# Autodesk Inventor assembly: entire arm
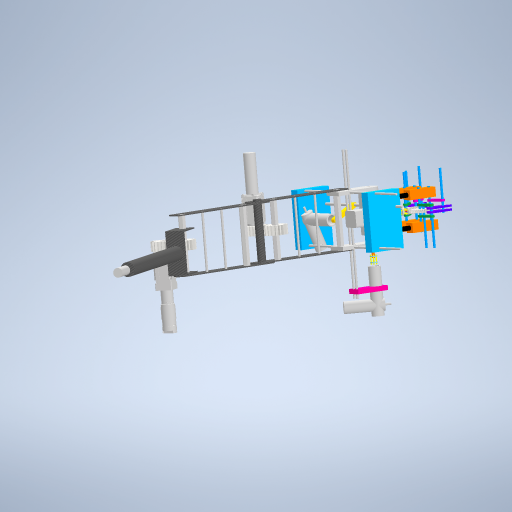
[picture p0: Inventor's stored thumbnail of the model, 512x512]
Saved by Autodesk Inventor 2023 (Build 270158000, 158)
## iProperties
Created: 2023-01-12
Part Number: entire arm
Document SubType Name: Assembly
Designer: victo
Author: victo
## Documents named in this file (3)
- C:\Users\victo\OneDrive\Documents\rcr\completely new\entire arm.iam
- C:\Users\victo\OneDrive\Documents\rcr\completely new\up to forearm full assembly.iam
- C:\Users\victo\OneDrive\Documents\rcr\completely new\Completed Klaw Mechanism (Fully Assembled).iam
## Components (2 placed, 2 different names)
1. up to forearm full assembly:1 [sub-assembly] — Mate:1, Mate:2, Mate:3, Flush:1
2. Completed Klaw Mechanism (Fully Assembled):1 [sub-assembly] — Mate:1, Mate:2, Mate:3, Flush:1
## Relationships (4: Mate 3, Flush 1)
- Mate:1: up to forearm full assembly:1 ↔ Completed Klaw Mechanism (Fully Assembled):1
- Mate:2: up to forearm full assembly:1 ↔ Completed Klaw Mechanism (Fully Assembled):1
- Mate:3: up to forearm full assembly:1 ↔ Completed Klaw Mechanism (Fully Assembled):1
- Flush:1 (-2.54 mm): up to forearm full assembly:1 ↔ Completed Klaw Mechanism (Fully Assembled):1
